# Autodesk Inventor assembly: bunny bot 2013 idea 1
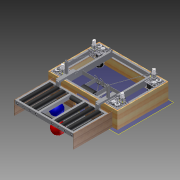
[picture p0: Inventor's stored thumbnail of the model, 180x180]
Saved by Autodesk Inventor 2012 (Build 160160000, 160)
## iProperties
Created: 2013-09-01
Part Number: bunny bot 2013 idea 1
Document SubType Name: Assembly
Designer: Bryce
Author: Bryce
## Documents named in this file (18)
- C:\Users\Bryce\Dropbox\Inventor Design Project Files\Independent Swerves\Inventor 2012\bunny bot 2013 idea 1.iam
- C:\Users\Bryce\Dropbox\Inventor Design Project Files\Independent Swerves\Inventor 2012\FULL SWERVE DRIVE ASSEMBLY!  2!.iam
- C:\Users\Bryce\Dropbox\Inventor Design Project Files\Independent Swerves\Inventor 2012\frame U 1 by 3.ipt
- C:\Users\Bryce\Dropbox\Inventor Design Project Files\Independent Swerves\Inventor 2012\frame U 1 by 3 long.ipt
- C:\Users\Bryce\Dropbox\Inventor Design Project Files\Independent Swerves\Inventor 2012\frame box 1 by 3.ipt
- C:\Users\Bryce\Dropbox\Inventor Design Project Files\Independent Swerves\Inventor 2012\plywood back pannel.ipt
- C:\Users\Bryce\Dropbox\Inventor Design Project Files\Independent Swerves\Inventor 2012\plywood side pannel.ipt
- C:\Users\Bryce\Dropbox\Inventor Design Project Files\Independent Swerves\Inventor 2012\bunny bot 2013 manipulator 2.iam
- C:\Users\Bryce\Dropbox\Inventor Design Project Files\Independent Swerves\Inventor 2012\manipulator apendage pivot.ipt
- C:\Users\Bryce\Dropbox\Inventor Design Project Files\Independent Swerves\Inventor 2012\manipulator spacer.ipt
- C:\Users\Bryce\Dropbox\Inventor Design Project Files\Independent Swerves\Inventor 2012\apendage arm.ipt
- C:\Users\Bryce\Dropbox\Inventor Design Project Files\Independent Swerves\Inventor 2012\plywood front pannel.ipt
- C:\Users\Bryce\Dropbox\Inventor Design Project Files\Independent Swerves\Inventor 2012\8 ball mechanism.iam
- C:\Users\Bryce\Dropbox\Inventor Design Project Files\Independent Swerves\Inventor 2012\dodge ball.ipt
- C:\Users\Bryce\Dropbox\Inventor Design Project Files\Independent Swerves\Inventor 2012\dodge ball squished.ipt
- C:\Users\Bryce\Dropbox\Inventor Design Project Files\Independent Swerves\Inventor 2012\pnumatic arm lever.ipt
- C:\Users\Bryce\Dropbox\Inventor Design Project Files\Independent Swerves\Inventor 2012\manipulator piston.ipt
- C:\Users\Bryce\Dropbox\Inventor Design Project Files\Independent Swerves\Inventor 2012\manipulator pnumaitic pivot.ipt
## Components (30 placed, 17 different names)
1. FULL SWERVE DRIVE ASSEMBLY!  2!:1 [sub-assembly] — Mate:6, Mate:7, Mate:8, Mate:23
2. FULL SWERVE DRIVE ASSEMBLY!  2!:2 [sub-assembly] — Mate:12, Mate:13, Mate:14
3. FULL SWERVE DRIVE ASSEMBLY!  2!:3 [sub-assembly] — Mate:9, Mate:10, Mate:11, Mate:24
4. FULL SWERVE DRIVE ASSEMBLY!  2!:4 [sub-assembly] — Mate:15, Mate:16, Mate:17, Mate:22
5. frame U 1 by 3:1 — Mate:1, Mate:2, Flush:1, Mate:5, Mate:14, Mate:15, Mate:27, Flush:11
6. frame U 1 by 3:2 — Mate:3, Mate:4, Flush:2, Flush:3, Mate:6, Mate:7, Mate:9, Mate:10, Flush:6, Mate:26, Flush:9
7. frame U 1 by 3 long:1 — Mate:1, Mate:4, Flush:3, Mate:5, Mate:11, Mate:12, Mate:13, Mate:25, Flush:7
8. frame U 1 by 3 long:2 — Mate:2, Mate:3, Flush:1, Flush:2, Mate:8, Mate:16, Mate:17, Mate:18, Mate:19, Flush:4, Mate:20, Mate:21, Flush:5, Flush:10, Mate:38, Mate:39, Flush:22, Mate:40, Mate:42, Mate:43, Flush:23
9. frame box 1 by 3:1 — Mate:18, Mate:19, Flush:4, Mate:29, Mate:41, Flush:24, Mate:52, Flush:28
10. frame box 1 by 3:2 — Mate:20, Mate:21, Flush:5, Mate:28, Flush:12, Mate:51, Flush:29
11. plywood back pannel:1 — Mate:25, Flush:6, Flush:7, Flush:8, Mate:53
12. plywood side pannel:1 — Mate:26, Flush:8, Flush:9
13. plywood side pannel:2 — Mate:27, Flush:10, Flush:11, Flush:21
14. bunny bot 2013 manipulator 2:1 [sub-assembly] — Mate:30, Mate:31, Flush:15, Flush:16, Flush:20
15. manipulator apendage pivot:1 — Mate:28, Flush:12, Flush:13, Mate:32, Mate:33, Mate:38
16. manipulator apendage pivot:2 — Flush:13, Mate:29, Mate:34, Mate:35, Flush:24
17. manipulator spacer:1 — Mate:30, Flush:15, Mate:36, Flush:17, Flush:18, Flush:20
18. manipulator spacer:2 — Mate:31, Flush:16, Flush:19, Mate:37
19. apendage arm:1 — Mate:32, Mate:33, Mate:36, Flush:17, Flush:18, Flush:26
20. apendage arm:2 — Mate:34, Mate:35, Flush:19, Mate:37, Mate:45, Flush:25, Mate:46
21. plywood front pannel:1 — Mate:39, Flush:21, Flush:22
22. 8 ball mechanism:1 [sub-assembly] — Mate:40, Mate:41, Mate:42
23. dodge ball:1 — Mate:43
24. dodge ball squished:1 — Flush:23
25. pnumatic arm lever:1 — Flush:26, Mate:48, Mate:50, Angle:1
26. pnumatic arm lever:2 — Mate:45, Flush:25, Mate:46, Mate:47, Mate:49, Angle:1
27. manipulator piston:1 — Mate:47, Mate:49, Mate:54, Angle:2
28. manipulator piston:2 — Mate:48, Mate:50, Mate:55, Angle:2
29. manipulator pnumaitic pivot:1 — Mate:52, Flush:28, Flush:30, Mate:53, Mate:54
30. manipulator pnumaitic pivot:2 — Mate:51, Flush:29, Flush:30, Mate:55
## Relationships (84: Mate 54, Flush 28, Angle 2)
- Mate:1: frame U 1 by 3:1 ↔ frame U 1 by 3 long:1
- Mate:2: frame U 1 by 3:1 ↔ frame U 1 by 3 long:2
- Mate:3: frame U 1 by 3:2 ↔ frame U 1 by 3 long:2
- Mate:4: frame U 1 by 3:2 ↔ frame U 1 by 3 long:1
- Flush:1: frame U 1 by 3:1 ↔ frame U 1 by 3 long:2
- Flush:2: frame U 1 by 3:2 ↔ frame U 1 by 3 long:2
- Flush:3: frame U 1 by 3:2 ↔ frame U 1 by 3 long:1
- Mate:5: frame U 1 by 3:1 ↔ frame U 1 by 3 long:1
- Mate:6: FULL SWERVE DRIVE ASSEMBLY!  2!:1 ↔ frame U 1 by 3:2
- Mate:7: FULL SWERVE DRIVE ASSEMBLY!  2!:1 ↔ frame U 1 by 3:2
- Mate:8: FULL SWERVE DRIVE ASSEMBLY!  2!:1 ↔ frame U 1 by 3 long:2
- Mate:9: FULL SWERVE DRIVE ASSEMBLY!  2!:3 ↔ frame U 1 by 3:2
- Mate:10: FULL SWERVE DRIVE ASSEMBLY!  2!:3 ↔ frame U 1 by 3:2
- Mate:11: FULL SWERVE DRIVE ASSEMBLY!  2!:3 ↔ frame U 1 by 3 long:1
- Mate:12: FULL SWERVE DRIVE ASSEMBLY!  2!:2 ↔ frame U 1 by 3 long:1
- Mate:13: FULL SWERVE DRIVE ASSEMBLY!  2!:2 ↔ frame U 1 by 3 long:1
- Mate:14: FULL SWERVE DRIVE ASSEMBLY!  2!:2 ↔ frame U 1 by 3:1
- Mate:15: FULL SWERVE DRIVE ASSEMBLY!  2!:4 ↔ frame U 1 by 3:1
- Mate:16: FULL SWERVE DRIVE ASSEMBLY!  2!:4 ↔ frame U 1 by 3 long:2
- Mate:17: FULL SWERVE DRIVE ASSEMBLY!  2!:4 ↔ frame U 1 by 3 long:2
- Mate:18: frame U 1 by 3 long:2 ↔ frame box 1 by 3:1
- Mate:19: frame U 1 by 3 long:2 ↔ frame box 1 by 3:1
- Flush:4: frame U 1 by 3 long:2 ↔ frame box 1 by 3:1
- Mate:20: frame U 1 by 3 long:2 ↔ frame box 1 by 3:2
- Mate:21: frame U 1 by 3 long:2 ↔ frame box 1 by 3:2
- Flush:5: frame U 1 by 3 long:2 ↔ frame box 1 by 3:2
- Mate:22: FULL SWERVE DRIVE ASSEMBLY!  2!:4
- Mate:23: FULL SWERVE DRIVE ASSEMBLY!  2!:1
- Mate:24: FULL SWERVE DRIVE ASSEMBLY!  2!:3
- Mate:25: frame U 1 by 3 long:1 ↔ plywood back pannel:1
- Flush:6: frame U 1 by 3:2 ↔ plywood back pannel:1
- Flush:7: frame U 1 by 3 long:1 ↔ plywood back pannel:1
- Mate:26: frame U 1 by 3:2 ↔ plywood side pannel:1
- Flush:8: plywood back pannel:1 ↔ plywood side pannel:1
- Flush:9: frame U 1 by 3:2 ↔ plywood side pannel:1
- Mate:27: frame U 1 by 3:1 ↔ plywood side pannel:2
- Flush:10: frame U 1 by 3 long:2 ↔ plywood side pannel:2
- Flush:11: frame U 1 by 3:1 ↔ plywood side pannel:2
- Mate:28: frame box 1 by 3:2 ↔ manipulator apendage pivot:1
- Flush:12 (-6.35 mm): frame box 1 by 3:2 ↔ manipulator apendage pivot:1
- Flush:13: manipulator apendage pivot:1 ↔ manipulator apendage pivot:2
- Mate:29: frame box 1 by 3:1 ↔ manipulator apendage pivot:2
- Mate:30: bunny bot 2013 manipulator 2:1 ↔ manipulator spacer:1
- Mate:31: bunny bot 2013 manipulator 2:1 ↔ manipulator spacer:2
- Flush:15: bunny bot 2013 manipulator 2:1 ↔ manipulator spacer:1
- Flush:16: bunny bot 2013 manipulator 2:1 ↔ manipulator spacer:2
- Mate:32: manipulator apendage pivot:1 ↔ apendage arm:1
- Mate:33 (3.175 mm): manipulator apendage pivot:1 ↔ apendage arm:1
- Mate:34: manipulator apendage pivot:2 ↔ apendage arm:2
- Mate:35 (3.175 mm): manipulator apendage pivot:2 ↔ apendage arm:2
- Mate:36: manipulator spacer:1 ↔ apendage arm:1
- Flush:17: manipulator spacer:1 ↔ apendage arm:1
- Flush:18: manipulator spacer:1 ↔ apendage arm:1
- Flush:19: manipulator spacer:2 ↔ apendage arm:2
- Mate:37: manipulator spacer:2 ↔ apendage arm:2
- Mate:38 (-165.1 mm): frame U 1 by 3 long:2 ↔ manipulator apendage pivot:1
- Flush:20 (104.775 mm): bunny bot 2013 manipulator 2:1 ↔ manipulator spacer:1
- Mate:39: frame U 1 by 3 long:2 ↔ plywood front pannel:1
- Flush:21: plywood side pannel:2 ↔ plywood front pannel:1
- Flush:22: frame U 1 by 3 long:2 ↔ plywood front pannel:1
- Mate:40: frame U 1 by 3 long:2 ↔ 8 ball mechanism:1
- Mate:41: frame box 1 by 3:1 ↔ 8 ball mechanism:1
- Mate:42: frame U 1 by 3 long:2 ↔ 8 ball mechanism:1
- Mate:43 (-164.7444 mm): frame U 1 by 3 long:2 ↔ dodge ball:1
- Flush:23 (97.4344 mm): frame U 1 by 3 long:2 ↔ dodge ball squished:1
- Flush:24 (-6.35 mm): frame box 1 by 3:1 ↔ manipulator apendage pivot:2
- Mate:45: apendage arm:2 ↔ pnumatic arm lever:2
- Flush:25 (25.4 mm): apendage arm:2 ↔ pnumatic arm lever:2
- Flush:26: apendage arm:1 ↔ pnumatic arm lever:1
- Mate:46 (88.9 mm): apendage arm:2 ↔ pnumatic arm lever:2
- Mate:47: pnumatic arm lever:2 ↔ manipulator piston:1
- Mate:48: pnumatic arm lever:1 ↔ manipulator piston:2
- Mate:49 (3.175 mm): pnumatic arm lever:2 ↔ manipulator piston:1
- Mate:50 (3.175 mm): pnumatic arm lever:1 ↔ manipulator piston:2
- Mate:51: frame box 1 by 3:2 ↔ manipulator pnumaitic pivot:2
- Mate:52: frame box 1 by 3:1 ↔ manipulator pnumaitic pivot:1
- Flush:28 (-3.175 mm): frame box 1 by 3:1 ↔ manipulator pnumaitic pivot:1
- Flush:29 (-3.175 mm): frame box 1 by 3:2 ↔ manipulator pnumaitic pivot:2
- Flush:30: manipulator pnumaitic pivot:1 ↔ manipulator pnumaitic pivot:2
- Mate:53 (-31.75 mm): plywood back pannel:1 ↔ manipulator pnumaitic pivot:1
- Mate:54: manipulator piston:1 ↔ manipulator pnumaitic pivot:1
- Mate:55: manipulator piston:2 ↔ manipulator pnumaitic pivot:2
- Angle:1 (0 deg): pnumatic arm lever:1 ↔ pnumatic arm lever:2
- Angle:2 (0 deg): manipulator piston:1 ↔ manipulator piston:2
